# Autodesk Inventor assembly: Assembly_Opentrons_Autofocus_v0
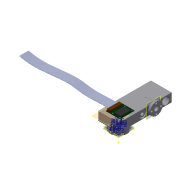
[picture p0: Inventor's stored thumbnail of the model, 180x180]
Saved by Autodesk Inventor 2019.4 (Build 234330000, 330)
## iProperties
Created: 2020-10-23
Part Number: Assembly_Opentrons_Autofocus_v0
Document SubType Name: Assembly
Designer: diederichbenedict
Author: diederichbenedict
## Documents named in this file (9)
- C:\Users\diederichbenedict\Dropbox\Dokumente\Promotion\PROJECTS\OPENTRONS\INVENTOR\Assembly_Opentrons_Autofocus_v0.iam
- C:\Users\diederichbenedict\Dropbox\Dokumente\Promotion\PROJECTS\OPENTRONS\INVENTOR\00_CCTV_Fisheye_Starlight_f2.8mm_Fno_1.4.ipt
- C:\Users\diederichbenedict\Dropbox\Dokumente\Promotion\PROJECTS\OPENTRONS\INVENTOR\00_Ringmagnet_25mm.ipt
- C:\Users\diederichbenedict\Dropbox\Dokumente\Promotion\PROJECTS\OPENTRONS\INVENTOR\01_Autofocus_CCTV12mm_spring_1.ipt
- C:\Users\diederichbenedict\Dropbox\Dokumente\Promotion\PROJECTS\OPENTRONS\INVENTOR\00_RasPi_Camera.ipt
- C:\Users\diederichbenedict\Dropbox\Dokumente\Promotion\PROJECTS\OPENTRONS\INVENTOR\01_Autofocus_Magnet_holder_v0.ipt
- C:\Users\diederichbenedict\Dropbox\Dokumente\Promotion\PROJECTS\OPENTRONS\INVENTOR\01_Slide_camera_x_v0.ipt
- C:\Users\diederichbenedict\Dropbox\Dokumente\Promotion\PROJECTS\OPENTRONS\INVENTOR\00_IGUS_Drylin_RJ4JP-01-06.ipt
- C:\Users\diederichbenedict\Dropbox\Dokumente\Promotion\PROJECTS\OPENTRONS\INVENTOR\00_spindel_slide.ipt
## Components (11 placed, 8 different names)
1. 00_RasPi_Camera:1 — Angle:2
2. 01_Autofocus_Magnet_holder_v0:1 — Insert:6
3. 00_IGUS_Drylin_RJ4JP-01-06:1
4. 00_spindel_slide:1 — Insert:5
5. 01_Slide_camera_x_v0:1 — Insert:5
6. 01_Autofocus_CCTV12mm_spring_1:3 — Insert:10, Insert:11
7. 01_Autofocus_CCTV12mm_spring_1:4 — Insert:9, Insert:10
8. 00_Ringmagnet_25mm:4 — Insert:8
9. 00_Ringmagnet_25mm:5 — Insert:7, Insert:8, Insert:9
10. 00_Ringmagnet_25mm:6 — Insert:6, Insert:7
11. 00_CCTV_Fisheye_Starlight_f2.8mm_Fno_1.4:1 — Insert:11
## Relationships (9: Insert 7, Angle 1, Flush 1)
- Angle:2 (0 deg): 00_RasPi_Camera:1
- [Flush]: 01_Autofocus_Magnet_holder_v0:1 ↔ 01_Slide_camera_x_v0:1
- Insert:5: 00_spindel_slide:1 ↔ 01_Slide_camera_x_v0:1
- Insert:6: 01_Autofocus_Magnet_holder_v0:1 ↔ 00_Ringmagnet_25mm:6
- Insert:7: 00_Ringmagnet_25mm:5 ↔ 00_Ringmagnet_25mm:6
- Insert:8: 00_Ringmagnet_25mm:4 ↔ 00_Ringmagnet_25mm:5
- Insert:9: 01_Autofocus_CCTV12mm_spring_1:4 ↔ 00_Ringmagnet_25mm:5
- Insert:10: 01_Autofocus_CCTV12mm_spring_1:3 ↔ 01_Autofocus_CCTV12mm_spring_1:4
- Insert:11 (-5 mm): 01_Autofocus_CCTV12mm_spring_1:3 ↔ 00_CCTV_Fisheye_Starlight_f2.8mm_Fno_1.4:1
## Named parameters: d13_d8 = 0 mm
